# Autodesk Inventor assembly: C2P2 Punching Machine
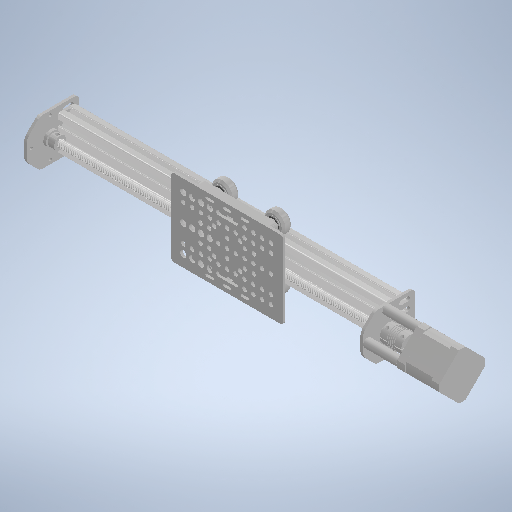
[picture p0: Inventor's stored thumbnail of the model, 512x512]
Saved by Autodesk Inventor 2025.2 (Build 292293000, 293)
## iProperties
Created: 2019-10-23
Part Number: C2P2 Punching Machine
Document SubType Name: Assembly
Designer: Johnson Ebenezer R
Author: Johnson Ebenezer R
## Documents named in this file (11)
- C:\Users\Simon\OneDrive\Desktop\Nema 17 V Slot Lead Screw Driven Actuator (2040 Al & Horizontal Gantry)\Threaded Rod Actuator (Horizontal Gantry).iam
- C:\Users\Simon\OneDrive\Desktop\Nema 17 V Slot Lead Screw Driven Actuator (2040 Al & Horizontal Gantry)\2040 Al Extrusion - Upper Middle Part (380mm).ipt
- C:\Users\Simon\OneDrive\Desktop\Nema 17 V Slot Lead Screw Driven Actuator (2040 Al & Horizontal Gantry)\Threaded Rod Plate Nema 17.ipt
- C:\Users\Simon\OneDrive\Desktop\Nema 17 V Slot Lead Screw Driven Actuator (2040 Al & Horizontal Gantry)\Nema 17 Stepper Motor.ipt
- C:\Users\Simon\OneDrive\Desktop\Nema 17 V Slot Lead Screw Driven Actuator (2040 Al & Horizontal Gantry)\Aluminum Spacer 1.5in.ipt
- C:\Users\Simon\OneDrive\Desktop\Nema 17 V Slot Lead Screw Driven Actuator (2040 Al & Horizontal Gantry)\Flexible Coupling 5mm x 8mm.ipt
- C:\Users\Simon\OneDrive\Desktop\Nema 17 V Slot Lead Screw Driven Actuator (2040 Al & Horizontal Gantry)\Lead Screw D8-P2-L400 (ACME).ipt
- C:\Users\Simon\OneDrive\Desktop\Nema 17 V Slot Lead Screw Driven Actuator (2040 Al & Horizontal Gantry)\Lead Screw Accessories\Ball Bearing 8 x 16 x 5.ipt
- C:\Users\Simon\OneDrive\Desktop\Nema 17 V Slot Lead Screw Driven Actuator (2040 Al & Horizontal Gantry)\Lead Screw Accessories\Lock Collar 8mm.ipt
- C:\Users\Simon\OneDrive\Desktop\Nema 17 V Slot Lead Screw Driven Actuator (2040 Al & Horizontal Gantry)\Lead Screw Accessories\Shim Washer 8mm.ipt
- C:\Users\Simon\OneDrive\Desktop\Nema 17 V Slot Lead Screw Driven Actuator (2040 Al & Horizontal Gantry)\V-Slot Gantry Kit Universal (for lead screw setup)\Gantry Kit (Horizontal).iam
## Components (16 placed, 10 different names)
1. 2040 Al Extrusion - Upper Middle Part (380mm):1 — Mate:12, Mate:13, Flush:12, Flush:15, Mate:41, Mate:42, Mate:43
2. Threaded Rod Plate Nema 17:1 — Mate:12, Flush:13, Flush:14, Mate:24, Mate:26, Mate:28, Flush:18
3. Threaded Rod Plate Nema 17:2 — Mate:13, Flush:12, Flush:14, Flush:15, Mate:14, Mate:15, Mate:16, Mate:17, Mate:18, Mate:19, Mate:27, Mate:29, Flush:13
4. Nema 17 Stepper Motor:1 — Mate:20, Mate:21, Mate:22, Mate:23, Flush:16
5. Aluminum Spacer 1.5in:1 — Mate:15, Mate:18, Mate:20
6. Aluminum Spacer 1.5in:2 — Mate:14, Mate:17, Mate:21
7. Aluminum Spacer 1.5in:3 — Mate:16, Mate:19, Mate:22
8. Flexible Coupling 5mm x 8mm:1 — Mate:23, Flush:16, Mate:25, Flush:17
9. Lead Screw D8-P2-L400 (ACME):1 — Mate:24, Mate:25, Mate:30, Mate:31, Mate:32, Mate:33, Mate:38, Mate:39, Flush:17, Mate:40, Rotation/Translation:1
10. Ball Bearing 8 x 16 x 5:1 — Mate:26, Mate:28, Mate:35
11. Ball Bearing 8 x 16 x 5:2 — Mate:27, Mate:29, Mate:34
12. Shim Washer 8mm:1 — Mate:32, Mate:35, Mate:36
13. Shim Washer 8mm:2 — Mate:33, Mate:34, Mate:37
14. Lock Collar 8mm:1 — Mate:30, Mate:36, Mate:38
15. Lock Collar 8mm:2 — Mate:31, Mate:37, Mate:39
16. Gantry Kit (Horizontal):1 [sub-assembly] — Mate:40, Flush:18, Rotation/Translation:1
## Relationships (40: Mate 32, Flush 7, RelateRotateTranslate 1)
- Mate:12: 2040 Al Extrusion - Upper Middle Part (380mm):1 ↔ Threaded Rod Plate Nema 17:1
- Mate:13: 2040 Al Extrusion - Upper Middle Part (380mm):1 ↔ Threaded Rod Plate Nema 17:2
- Flush:12 (-4 mm): 2040 Al Extrusion - Upper Middle Part (380mm):1 ↔ Threaded Rod Plate Nema 17:2
- Flush:13: Threaded Rod Plate Nema 17:1 ↔ Threaded Rod Plate Nema 17:2
- Flush:14: Threaded Rod Plate Nema 17:1 ↔ Threaded Rod Plate Nema 17:2
- Flush:15 (-6.5 mm): 2040 Al Extrusion - Upper Middle Part (380mm):1 ↔ Threaded Rod Plate Nema 17:2
- Mate:14: Threaded Rod Plate Nema 17:2 ↔ Aluminum Spacer 1.5in:2
- Mate:15: Threaded Rod Plate Nema 17:2 ↔ Aluminum Spacer 1.5in:1
- Mate:16: Threaded Rod Plate Nema 17:2 ↔ Aluminum Spacer 1.5in:3
- Mate:17: Threaded Rod Plate Nema 17:2 ↔ Aluminum Spacer 1.5in:2
- Mate:18: Threaded Rod Plate Nema 17:2 ↔ Aluminum Spacer 1.5in:1
- Mate:19: Threaded Rod Plate Nema 17:2 ↔ Aluminum Spacer 1.5in:3
- Mate:20: Nema 17 Stepper Motor:1 ↔ Aluminum Spacer 1.5in:1
- Mate:21: Nema 17 Stepper Motor:1 ↔ Aluminum Spacer 1.5in:2
- Mate:22: Nema 17 Stepper Motor:1 ↔ Aluminum Spacer 1.5in:3
- Mate:23: Nema 17 Stepper Motor:1 ↔ Flexible Coupling 5mm x 8mm:1
- Flush:16: Nema 17 Stepper Motor:1 ↔ Flexible Coupling 5mm x 8mm:1
- Mate:24: Threaded Rod Plate Nema 17:1 ↔ Lead Screw D8-P2-L400 (ACME):1
- Mate:25: Flexible Coupling 5mm x 8mm:1 ↔ Lead Screw D8-P2-L400 (ACME):1
- Mate:26: Threaded Rod Plate Nema 17:1 ↔ Ball Bearing 8 x 16 x 5:1
- Mate:27: Threaded Rod Plate Nema 17:2 ↔ Ball Bearing 8 x 16 x 5:2
- Mate:28: Threaded Rod Plate Nema 17:1 ↔ Ball Bearing 8 x 16 x 5:1
- Mate:29: Threaded Rod Plate Nema 17:2 ↔ Ball Bearing 8 x 16 x 5:2
- Mate:30: Lead Screw D8-P2-L400 (ACME):1 ↔ Lock Collar 8mm:1
- Mate:31: Lead Screw D8-P2-L400 (ACME):1 ↔ Lock Collar 8mm:2
- Mate:32: Lead Screw D8-P2-L400 (ACME):1 ↔ Shim Washer 8mm:1
- Mate:33: Lead Screw D8-P2-L400 (ACME):1 ↔ Shim Washer 8mm:2
- Mate:34: Ball Bearing 8 x 16 x 5:2 ↔ Shim Washer 8mm:2
- Mate:35: Ball Bearing 8 x 16 x 5:1 ↔ Shim Washer 8mm:1
- Mate:36: Shim Washer 8mm:1 ↔ Lock Collar 8mm:1
- Mate:37: Shim Washer 8mm:2 ↔ Lock Collar 8mm:2
- Mate:38: Lead Screw D8-P2-L400 (ACME):1 ↔ Lock Collar 8mm:1
- Mate:39: Lead Screw D8-P2-L400 (ACME):1 ↔ Lock Collar 8mm:2
- Flush:17: Flexible Coupling 5mm x 8mm:1 ↔ Lead Screw D8-P2-L400 (ACME):1
- Mate:40: Lead Screw D8-P2-L400 (ACME):1 ↔ Gantry Kit (Horizontal):1
- Flush:18: Threaded Rod Plate Nema 17:1 ↔ Gantry Kit (Horizontal):1
- Rotation/Translation:1 [RelateRotateTranslate] (25.133 mm): Lead Screw D8-P2-L400 (ACME):1 ↔ Gantry Kit (Horizontal):1
- Mate:41: 2040 Al Extrusion - Upper Middle Part (380mm):1
- Mate:42: 2040 Al Extrusion - Upper Middle Part (380mm):1
- Mate:43: 2040 Al Extrusion - Upper Middle Part (380mm):1
